# Autodesk Inventor assembly: Mold Design1
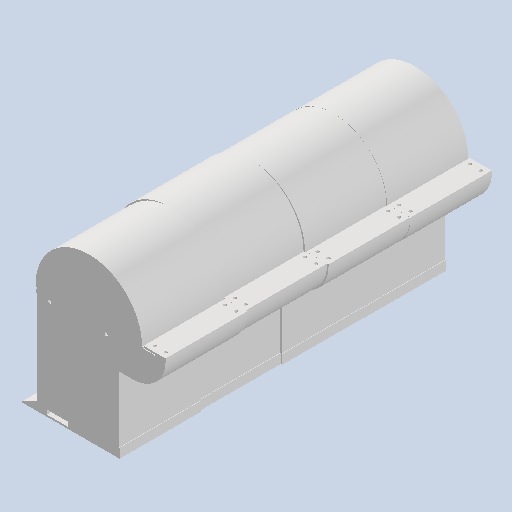
[picture p0: Inventor's stored thumbnail of the model, 512x512]
Saved by Autodesk Inventor 2025 (Build 290162000, 162)
## iProperties
Created: 2025-08-28
Part Number: Mold Design1
Document SubType Name: Assembly
Designer: Pravoslav
Author: Pravoslav
## Documents named in this file (6)
- D:\Škola\VUT\Igem\šachta\taker\dávkovanie\konnst\Mold Design1.iam
- D:\Škola\VUT\Igem\šachta\taker\dávkovanie\konnst\bottom.ipt
- D:\Škola\VUT\Igem\šachta\taker\dávkovanie\konnst\Low.ipt
- D:\Škola\VUT\Igem\šachta\taker\dávkovanie\konnst\Holder.ipt
- D:\Škola\VUT\Igem\šachta\taker\dávkovanie\konnst\coupol.ipt
- D:\Škola\VUT\Igem\šachta\taker\dávkovanie\konnst\cap.ipt
## Components (20 placed, 5 different names)
1. bottom:1 — Mate:1, Mate:17
2. Low:1 — Mate:1, Mate:2
3. Holder:1 — Mate:2, Mate:3, Mate:4
4. coupol:1 — Mate:3
5. cap:1 — Mate:4
6. bottom:3 — Mate:17, Mate:27
7. Low:3
8. Holder:3
9. coupol:3
10. cap:3
11. bottom:4 — Mate:27, Mate:28
12. Low:4
13. Holder:4
14. coupol:4
15. cap:4
16. bottom:5 — Mate:28
17. Low:5
18. Holder:5
19. coupol:5
20. cap:5
## Relationships (20: Mate 20)
- Mate:1: bottom:1 ↔ Low:1
- Mate:2: Low:1 ↔ Holder:1
- Mate:3: Holder:1 ↔ coupol:1
- Mate:4: Holder:1 ↔ cap:1
- [Mate]: bottom:3 ↔ Low:3
- [Mate]: Low:3 ↔ Holder:3
- [Mate]: Holder:3 ↔ coupol:3
- [Mate]: Holder:3 ↔ cap:3
- Mate:17: bottom:1 ↔ bottom:3
- [Mate]: bottom:4 ↔ Low:4
- [Mate]: Low:4 ↔ Holder:4
- [Mate]: Holder:4 ↔ coupol:4
- [Mate]: Holder:4 ↔ cap:4
- [Mate]: bottom:5 ↔ Low:5
- [Mate]: Low:5 ↔ Holder:5
- [Mate]: Holder:5 ↔ coupol:5
- [Mate]: Holder:5 ↔ cap:5
- [Mate]: bottom:4 ↔ bottom:5
- Mate:27: bottom:3 ↔ bottom:4
- Mate:28: bottom:4 ↔ bottom:5
## Named parameters: d8_d0 = 0 mm, d9_d1 = 0 mm, d10_d2 = 0 mm, d11_d3 = 0 mm, d17_d0 = 0 mm, d18_d1 = 0 mm, d19_d2 = 0 mm, d20_d3 = 0 mm, d21_d8_d0 = 0 mm, d22_d9_d1 = 0 mm, d23_d10_d2 = 0 mm, d24_d11_d3 = 0 mm, d25_d16 = 0 mm
